# Autodesk Inventor assembly: turret assembly
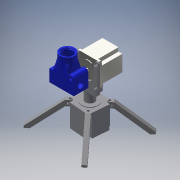
[picture p0: Inventor's stored thumbnail of the model, 180x180]
Saved by Autodesk Inventor 2019 (Build 230136000, 136)
## iProperties
Created: 2022-03-28
Part Number: turret assembly
Document SubType Name: Assembly
Designer: Ian
Author: Ian
## Documents named in this file (12)
- D:\Ian\Documents\Projects\autoturret\mechanical design\turret assembly.iam
- D:\Ian\Documents\Projects\autoturret\mechanical design\norm bottle.iam
- D:\Ian\Documents\Projects\autoturret\mechanical design\brake line.ipt
- D:\Ian\Documents\Projects\autoturret\mechanical design\bottle clamp.ipt
- D:\Ian\Documents\Projects\autoturret\mechanical design\wierd bearing interface part.ipt
- D:\Ian\Documents\Projects\autoturret\mechanical design\608 skate bearing.ipt
- D:\Ian\Documents\Projects\autoturret\mechanical design\left stand.ipt
- D:\Ian\Documents\Projects\autoturret\mechanical design\base thingy.ipt
- D:\Ian\Documents\Projects\autoturret\mechanical design\Gun Body 04-02-2022.ipt
- D:\Ian\Documents\Projects\autoturret\mechanical design\Big Chungus Motor.ipt
- D:\Ian\Documents\Projects\autoturret\mechanical design\Gimbal Arm.ipt
- D:\Ian\Documents\Projects\autoturret\mechanical design\Foot thing.ipt
## Components (18 placed, 11 different names)
1. norm bottle:1 [sub-assembly] — Insert:1
2. brake line:1 — Insert:1
3. bottle clamp:1 — Flush:1, Mate:1, Flush:2, Mate:2, Flush:3, Flush:4
4. wierd bearing interface part:1 — Flush:1, Mate:1, Flush:2, Insert:2
5. wierd bearing interface part:2 — Mate:2, Flush:3, Flush:4, Insert:3
6. 608 skate bearing:1 — Insert:3, Insert:4
7. 608 skate bearing:2 — Insert:2, Flush:5, Flush:6
8. left stand:1 — Flush:5, Flush:6, Flush:7, Flush:8
9. left stand:2 — Insert:4, Flush:7, Flush:9
10. base thingy:1 — Flush:8, Flush:9
11. Gun Body 04-02-2022:1 — Mate:4, Mate:5
12. Big Chungus Motor:1 — Mate:4, Mate:5, Flush:10
13. Gimbal Arm:1 — Flush:10, Mate:6, Mate:7
14. Big Chungus Motor:2 — Mate:6, Mate:7, Mate:8, Mate:9, Angle:1, Mate:10, Mate:11, Mate:12, Mate:13, Mate:14, Mate:15, Angle:2, Angle:3, Angle:4
15. Foot thing:1 — Mate:8, Mate:9, Angle:1
16. Foot thing:2 — Mate:11, Mate:14, Angle:3
17. Foot thing:3 — Mate:10, Mate:13, Angle:4
18. Foot thing:4 — Mate:12, Mate:15, Angle:2
## Relationships (32: Mate 14, Flush 10, Insert 4, Angle 4)
- Insert:1 (-40 mm): norm bottle:1 ↔ brake line:1
- Flush:1: bottle clamp:1 ↔ wierd bearing interface part:1
- Mate:1 (2 mm): bottle clamp:1 ↔ wierd bearing interface part:1
- Flush:2: bottle clamp:1 ↔ wierd bearing interface part:1
- Mate:2 (2 mm): bottle clamp:1 ↔ wierd bearing interface part:2
- Flush:3: bottle clamp:1 ↔ wierd bearing interface part:2
- Flush:4: bottle clamp:1 ↔ wierd bearing interface part:2
- Insert:2: wierd bearing interface part:1 ↔ 608 skate bearing:2
- Insert:3: wierd bearing interface part:2 ↔ 608 skate bearing:1
- Flush:5: 608 skate bearing:2 ↔ left stand:1
- Flush:6: 608 skate bearing:2 ↔ left stand:1
- Insert:4: 608 skate bearing:1 ↔ left stand:2
- Flush:7: left stand:1 ↔ left stand:2
- Flush:8: left stand:1 ↔ base thingy:1
- Flush:9: left stand:2 ↔ base thingy:1
- Mate:4: Gun Body 04-02-2022:1 ↔ Big Chungus Motor:1
- Mate:5: Gun Body 04-02-2022:1 ↔ Big Chungus Motor:1
- Flush:10: Big Chungus Motor:1 ↔ Gimbal Arm:1
- Mate:6: Gimbal Arm:1 ↔ Big Chungus Motor:2
- Mate:7: Gimbal Arm:1 ↔ Big Chungus Motor:2
- Mate:8: Big Chungus Motor:2 ↔ Foot thing:1
- Mate:9: Big Chungus Motor:2 ↔ Foot thing:1
- Angle:1 (-45 deg): Big Chungus Motor:2 ↔ Foot thing:1
- Mate:10: Big Chungus Motor:2 ↔ Foot thing:3
- Mate:11: Big Chungus Motor:2 ↔ Foot thing:2
- Mate:12: Big Chungus Motor:2 ↔ Foot thing:4
- Mate:13: Big Chungus Motor:2 ↔ Foot thing:3
- Mate:14: Big Chungus Motor:2 ↔ Foot thing:2
- Mate:15: Big Chungus Motor:2 ↔ Foot thing:4
- Angle:2 (-45 deg): Big Chungus Motor:2 ↔ Foot thing:4
- Angle:3 (135 deg): Big Chungus Motor:2 ↔ Foot thing:2
- Angle:4 (45 deg): Big Chungus Motor:2 ↔ Foot thing:3
